# Autodesk Inventor assembly: Ensamblaje1
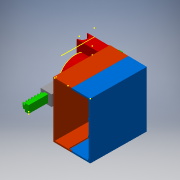
[picture p0: Inventor's stored thumbnail of the model, 180x180]
Saved by Autodesk Inventor 2018.2 (Build 222227000, 227)
## iProperties
Created: 2016-04-06
Part Number: Ensamblaje1
Material: Genérico
Document SubType Name: Assembly
Designer: Usuario
Mass: 591.4 g
Surface Area: 1727.06 cm^2
Volume: 591.4 cm^3
Density: 1 g/cm^3
Author: Usuario
## Documents named in this file (7)
- D:\DESKTOP\carrera\3º carrera\segundo cuatrimestre\robotica\ROBOTICO\DESIGN\Ensamblaje1.iam
- D:\DESKTOP\carrera\3º carrera\segundo cuatrimestre\robotica\ROBOTICO\DESIGN\cilindro.ipt
- D:\DESKTOP\carrera\3º carrera\segundo cuatrimestre\robotica\ROBOTICO\DESIGN\cremallera.ipt
- D:\DESKTOP\carrera\3º carrera\segundo cuatrimestre\robotica\ROBOTICO\DESIGN\engranaje.ipt
- D:\DESKTOP\carrera\3º carrera\segundo cuatrimestre\robotica\ROBOTICO\DESIGN\base sup.ipt
- D:\DESKTOP\carrera\3º carrera\segundo cuatrimestre\robotica\ROBOTICO\DESIGN\base inf.ipt
- D:\DESKTOP\carrera\3º carrera\segundo cuatrimestre\robotica\ROBOTICO\DESIGN\SOPORTE FINAL.ipt
## Components (6 placed, 6 different names)
1. cilindro:1 — Coincidencia:16, Nivelación:5, Coincidencia:17, Coincidencia:18
2. cremallera:1 — Coincidencia:14, Nivelación:2, Coincidencia:19, Coincidencia:20
3. engranaje:1 — Coincidencia:14, Nivelación:2
4. base sup:1 — Nivelación:3, Nivelación:4, Coincidencia:15, Coincidencia:16, Nivelación:5
5. base inf:1 — Nivelación:3, Nivelación:4, Coincidencia:15
6. SOPORTE FINAL:1 — Coincidencia:17, Coincidencia:18, Coincidencia:19, Coincidencia:20
## Relationships (11: Mate 7, Flush 4)
- Coincidencia:14 [Mate]: cremallera:1 ↔ engranaje:1
- Nivelación:2 [Flush]: cremallera:1 ↔ engranaje:1
- Nivelación:3 [Flush]: base sup:1 ↔ base inf:1
- Nivelación:4 [Flush]: base sup:1 ↔ base inf:1
- Coincidencia:15 [Mate]: base sup:1 ↔ base inf:1
- Coincidencia:16 [Mate]: cilindro:1 ↔ base sup:1
- Nivelación:5 [Flush]: cilindro:1 ↔ base sup:1
- Coincidencia:17 [Mate]: cilindro:1 ↔ SOPORTE FINAL:1
- Coincidencia:18 [Mate]: cilindro:1 ↔ SOPORTE FINAL:1
- Coincidencia:19 [Mate]: cremallera:1 ↔ SOPORTE FINAL:1
- Coincidencia:20 [Mate]: cremallera:1 ↔ SOPORTE FINAL:1
